# Autodesk Inventor assembly: Marco_apm_002-1
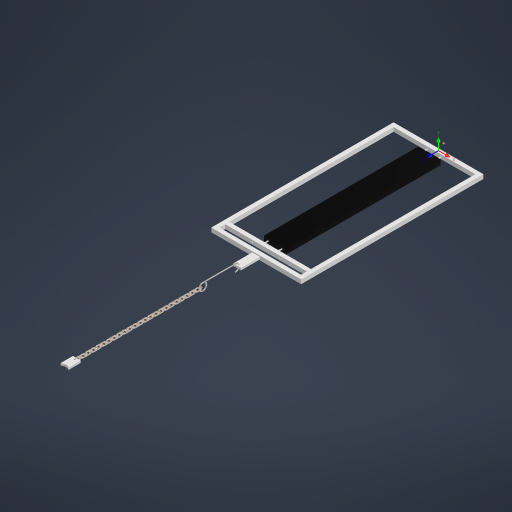
[picture p0: Inventor's stored thumbnail of the model, 512x512]
Saved by Autodesk Inventor 2024 (Build 280153000, 153)
## iProperties
Created: 2023-05-13
Part Number: Marco_apm_002-1
Document SubType Name: Assembly
Designer: javie
Author: javie
## Documents named in this file (7)
- C:\Users\javie\Downloads\Piezas CMR\Marco_APM_002\Marco_apm_002-2.iam
- C:\Users\javie\Downloads\Piezas CMR\Marco_Conveyor_Aereo.iam
- C:\Users\javie\Downloads\Piezas CMR\Marco_APM_002\Piezas\APM_002-2.ipt
- C:\Users\javie\Downloads\Piezas CMR\Marcos_solids\Topes_apm_002-2.ipt
- C:\Users\javie\Downloads\Piezas CMR\Marcos_solids\S_horizontal.ipt
- C:\Users\javie\Downloads\Piezas CMR\Marcos_solids\Pieza3.ipt
- C:\Users\javie\Downloads\Piezas CMR\S_RobotStudio_Model\Pieza2.ipt
## Components (7 placed, 6 different names)
1. Marco_Conveyor_Aereo:1 [sub-assembly] — Nivelación:3, Insertar:7, Nivelación:4, Nivelación:5
2. APM_002-2:1 — Insertar:4, Insertar:5, Insertar:6
3. S_horizontal:2 — Insertar:2, Insertar:3
4. Topes_apm_002-2:2 — Insertar:2, Insertar:3, Insertar:4
5. Pieza3:1 — Nivelación:3
6. Topes_apm_002-2:3 — Insertar:5, Insertar:6, Insertar:7
7. Pieza2:1 — Nivelación:4, Nivelación:5
## Relationships (9: Insert 6, Flush 3)
- Insertar:2: S_horizontal:2 ↔ Topes_apm_002-2:2
- Insertar:3: S_horizontal:2 ↔ Topes_apm_002-2:2
- Insertar:4: APM_002-2:1 ↔ Topes_apm_002-2:2
- Nivelación:3 [Flush]: Marco_Conveyor_Aereo:1 ↔ Pieza3:1
- Insertar:5: APM_002-2:1 ↔ Topes_apm_002-2:3
- Insertar:6: APM_002-2:1 ↔ Topes_apm_002-2:3
- Insertar:7: Marco_Conveyor_Aereo:1 ↔ Topes_apm_002-2:3
- Nivelación:4 [Flush]: Marco_Conveyor_Aereo:1 ↔ Pieza2:1
- Nivelación:5 [Flush]: Marco_Conveyor_Aereo:1 ↔ Pieza2:1
